# Autodesk Inventor assembly: GP6-100
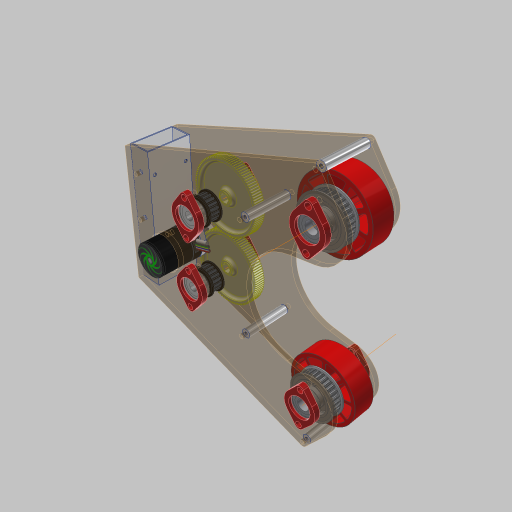
[picture p0: Inventor's stored thumbnail of the model, 512x512]
Saved by Autodesk Inventor 2023.5 (Build 275446000, 446)
## iProperties
Created: 2025-02-23
Part Number: GP6-100
Document SubType Name: Assembly
Designer: slick
Author: slick
## Documents named in this file (16)
- C:\Users\slick\OneDrive\Desktop\2025-ReefScape---CAD\Gripper\GP6\GP6-100.iam
- C:\Users\slick\OneDrive\Desktop\2025-ReefScape---CAD\Gripper\GP6\GP6-001.ipt
- C:\Users\slick\OneDrive\Desktop\2025-ReefScape---CAD\Gripper\GP6\GP6-003.ipt
- C:\Users\slick\OneDrive\Desktop\2025-ReefScape---CAD\Gripper\GP6\GP6-002.ipt
- C:\Users\slick\OneDrive\Desktop\2025-ReefScape---CAD\COMMON PARTS\BEARINGS\0_500_ID_x_1_125_OD_x_0_313_WD_Flanged_Bearing_217-2731.ipt
- C:\Users\slick\OneDrive\Desktop\2025-ReefScape---CAD\COMMON PARTS\BEARINGS\Bearing Retainer\Retainer.ipt
- C:\Users\slick\OneDrive\Desktop\2025-ReefScape---CAD\COMMON PARTS\BEARINGS\0_375_ID_x_1_125_OD_x_0_313_WD_Flanged_Bearing_217-2732.ipt
- C:\Users\slick\OneDrive\Desktop\2025-ReefScape---CAD\Gripper\GP6\GP6-005.ipt
- C:\Users\slick\OneDrive\Desktop\2025-ReefScape---CAD\COMMON PARTS\MOTORS\Minion.ipt
- C:\Users\slick\OneDrive\Desktop\2025-ReefScape---CAD\Gripper\GP6\GP6-006.ipt
- C:\Users\slick\OneDrive\Desktop\2025-ReefScape---CAD\COMMON PARTS\GEARS\15t Spur Gear\15t Spur Gear.ipt
- C:\Users\slick\OneDrive\Desktop\2025-ReefScape---CAD\COMMON PARTS\GEARS\32 dp gear\100t_Aluminum_Spur_Gear_32_DP_3_8_Hex_Bore_217-5865.ipt
- C:\Users\slick\OneDrive\Desktop\2025-ReefScape---CAD\Gripper\GP6\GP6-007.ipt
- C:\Users\slick\OneDrive\Desktop\2025-ReefScape---CAD\COMMON PARTS\PULLEYS\htd\30t_x_9mm_Wide_Double_Flange_Aluminum_Pulley_HTD_5mm_1_2_Hex_Bore_217-3229.ipt
- C:\Users\slick\OneDrive\Desktop\2025-ReefScape---CAD\COMMON PARTS\PULLEYS\htd\18t_x_9mm_Wide_Double_Flange_Aluminum_Pulley_HTD_5mm_1_2_Hex_Bore_217-3225.ipt
- C:\Users\slick\OneDrive\Desktop\2025-ReefScape---CAD\COMMON PARTS\WHEELS\am-3946 3IN 375Hex Compliant Wheel REV 3.ipt
## Components (35 placed, 15 different names)
1. GP6-001:1 — Insert:1, Insert:2, Insert:35, Insert:36, Insert:41, Insert:42, Insert:43, Insert:46, Insert:47, Insert:54, Insert:55, Insert:60, Insert:61, Insert:62, Insert:63
2. GP6-003:1 — Insert:1, Insert:2, Insert:3, Insert:4
3. GP6-002:1 — Insert:3, Insert:4, Insert:38, Insert:39, Insert:40, Insert:44, Insert:45, Insert:48, Insert:49, Insert:50, Insert:51, Insert:52, Insert:53, Insert:56, Insert:57, Insert:58, Insert:59
4. GP6-005:1 — Insert:31, Insert:32, Insert:33, Insert:34
5. Minion:1 — Insert:31, Insert:32, Insert:37
6. GP6-006:1 — Insert:33, Insert:35
7. GP6-006:2 — Insert:34, Insert:36
8. 15t Spur Gear:1 — Insert:37
9. 100t_Aluminum_Spur_Gear_32_DP_3_8_Hex_Bore_217-5865:1 — Flush:1, Mate:12, Mate:15
10. 100t_Aluminum_Spur_Gear_32_DP_3_8_Hex_Bore_217-5865:2 — Flush:1, Mate:14
11. GP6-007:1 — Insert:38
12. GP6-007:2 — Insert:40
13. GP6-007:3 — Insert:41
14. GP6-007:4 — Insert:39
15. 30t_x_9mm_Wide_Double_Flange_Aluminum_Pulley_HTD_5mm_1_2_Hex_Bore_217-3229:1 — Flush:2, Flush:4, Mate:9, Mate:10
16. 30t_x_9mm_Wide_Double_Flange_Aluminum_Pulley_HTD_5mm_1_2_Hex_Bore_217-3229:2 — Flush:3, Flush:4, Mate:17, Mate:18
17. 18t_x_9mm_Wide_Double_Flange_Aluminum_Pulley_HTD_5mm_1_2_Hex_Bore_217-3225:1 — Flush:2, Mate:11, Mate:12
18. 18t_x_9mm_Wide_Double_Flange_Aluminum_Pulley_HTD_5mm_1_2_Hex_Bore_217-3225:2 — Flush:3, Mate:13, Mate:14, Mate:16
19. am-3946 3IN 375Hex Compliant Wheel REV 3:1 — Mate:9, Flush:5
20. am-3946 3IN 375Hex Compliant Wheel REV 3:4 — Mate:18, Flush:5
21. 0_500_ID_x_1_125_OD_x_0_313_WD_Flanged_Bearing_217-2731:1 — Insert:45, Mate:10
22. 0_500_ID_x_1_125_OD_x_0_313_WD_Flanged_Bearing_217-2731:2 — Insert:42
23. 0_500_ID_x_1_125_OD_x_0_313_WD_Flanged_Bearing_217-2731:3 — Insert:43
24. 0_500_ID_x_1_125_OD_x_0_313_WD_Flanged_Bearing_217-2731:4 — Insert:44, Mate:17
25. 0_375_ID_x_1_125_OD_x_0_313_WD_Flanged_Bearing_217-2732:1 — Insert:46, Mate:15
26. 0_375_ID_x_1_125_OD_x_0_313_WD_Flanged_Bearing_217-2732:2 — Insert:49, Mate:11
27. 0_375_ID_x_1_125_OD_x_0_313_WD_Flanged_Bearing_217-2732:3 — Insert:48, Mate:13, Mate:16
28. 0_375_ID_x_1_125_OD_x_0_313_WD_Flanged_Bearing_217-2732:4 — Insert:47
29. Retainer:1 — Insert:50, Insert:51
30. Retainer:2 — Insert:52, Insert:53
31. Retainer:3 — Insert:54, Insert:55
32. Retainer:4 — Insert:56, Insert:57
33. Retainer:5 — Insert:58, Insert:59
34. Retainer:6 — Insert:62, Insert:63
35. Retainer:7 — Insert:60, Insert:61
## Relationships (52: Insert 37, Mate 10, Flush 5)
- Insert:1: GP6-001:1 ↔ GP6-003:1
- Insert:2: GP6-001:1 ↔ GP6-003:1
- Insert:3: GP6-003:1 ↔ GP6-002:1
- Insert:4: GP6-003:1 ↔ GP6-002:1
- Insert:31: GP6-005:1 ↔ Minion:1
- Insert:32: GP6-005:1 ↔ Minion:1
- Insert:33: GP6-005:1 ↔ GP6-006:1
- Insert:34: GP6-005:1 ↔ GP6-006:2
- Insert:35: GP6-001:1 ↔ GP6-006:1
- Insert:36: GP6-001:1 ↔ GP6-006:2
- Insert:37: Minion:1 ↔ 15t Spur Gear:1
- Flush:1: 100t_Aluminum_Spur_Gear_32_DP_3_8_Hex_Bore_217-5865:1 ↔ 100t_Aluminum_Spur_Gear_32_DP_3_8_Hex_Bore_217-5865:2
- Insert:38: GP6-002:1 ↔ GP6-007:1
- Insert:39: GP6-002:1 ↔ GP6-007:4
- Insert:40: GP6-002:1 ↔ GP6-007:2
- Insert:41: GP6-001:1 ↔ GP6-007:3
- Flush:2: 30t_x_9mm_Wide_Double_Flange_Aluminum_Pulley_HTD_5mm_1_2_Hex_Bore_217-3229:1 ↔ 18t_x_9mm_Wide_Double_Flange_Aluminum_Pulley_HTD_5mm_1_2_Hex_Bore_217-3225:1
- Flush:3: 30t_x_9mm_Wide_Double_Flange_Aluminum_Pulley_HTD_5mm_1_2_Hex_Bore_217-3229:2 ↔ 18t_x_9mm_Wide_Double_Flange_Aluminum_Pulley_HTD_5mm_1_2_Hex_Bore_217-3225:2
- Flush:4: 30t_x_9mm_Wide_Double_Flange_Aluminum_Pulley_HTD_5mm_1_2_Hex_Bore_217-3229:1 ↔ 30t_x_9mm_Wide_Double_Flange_Aluminum_Pulley_HTD_5mm_1_2_Hex_Bore_217-3229:2
- Mate:9: 30t_x_9mm_Wide_Double_Flange_Aluminum_Pulley_HTD_5mm_1_2_Hex_Bore_217-3229:1 ↔ am-3946 3IN 375Hex Compliant Wheel REV 3:1
- Insert:42: GP6-001:1 ↔ 0_500_ID_x_1_125_OD_x_0_313_WD_Flanged_Bearing_217-2731:2
- Insert:43: GP6-001:1 ↔ 0_500_ID_x_1_125_OD_x_0_313_WD_Flanged_Bearing_217-2731:3
- Insert:44: GP6-002:1 ↔ 0_500_ID_x_1_125_OD_x_0_313_WD_Flanged_Bearing_217-2731:4
- Insert:45: GP6-002:1 ↔ 0_500_ID_x_1_125_OD_x_0_313_WD_Flanged_Bearing_217-2731:1
- Insert:46: GP6-001:1 ↔ 0_375_ID_x_1_125_OD_x_0_313_WD_Flanged_Bearing_217-2732:1
- Insert:47: GP6-001:1 ↔ 0_375_ID_x_1_125_OD_x_0_313_WD_Flanged_Bearing_217-2732:4
- Insert:48: GP6-002:1 ↔ 0_375_ID_x_1_125_OD_x_0_313_WD_Flanged_Bearing_217-2732:3
- Insert:49: GP6-002:1 ↔ 0_375_ID_x_1_125_OD_x_0_313_WD_Flanged_Bearing_217-2732:2
- Insert:50: GP6-002:1 ↔ Retainer:1
- Insert:51: GP6-002:1 ↔ Retainer:1
- Insert:52: GP6-002:1 ↔ Retainer:2
- Insert:53: GP6-002:1 ↔ Retainer:2
- Insert:54: GP6-001:1 ↔ Retainer:3
- Insert:55: GP6-001:1 ↔ Retainer:3
- Insert:56: GP6-002:1 ↔ Retainer:4
- Insert:57: GP6-002:1 ↔ Retainer:4
- Insert:58: GP6-002:1 ↔ Retainer:5
- Insert:59: GP6-002:1 ↔ Retainer:5
- Insert:60: GP6-001:1 ↔ Retainer:7
- Insert:61: GP6-001:1 ↔ Retainer:7
- Insert:62: GP6-001:1 ↔ Retainer:6
- Insert:63: GP6-001:1 ↔ Retainer:6
- Mate:10: 30t_x_9mm_Wide_Double_Flange_Aluminum_Pulley_HTD_5mm_1_2_Hex_Bore_217-3229:1 ↔ 0_500_ID_x_1_125_OD_x_0_313_WD_Flanged_Bearing_217-2731:1
- Mate:11: 18t_x_9mm_Wide_Double_Flange_Aluminum_Pulley_HTD_5mm_1_2_Hex_Bore_217-3225:1 ↔ 0_375_ID_x_1_125_OD_x_0_313_WD_Flanged_Bearing_217-2732:2
- Mate:12: 100t_Aluminum_Spur_Gear_32_DP_3_8_Hex_Bore_217-5865:1 ↔ 18t_x_9mm_Wide_Double_Flange_Aluminum_Pulley_HTD_5mm_1_2_Hex_Bore_217-3225:1
- Mate:13: 18t_x_9mm_Wide_Double_Flange_Aluminum_Pulley_HTD_5mm_1_2_Hex_Bore_217-3225:2 ↔ 0_375_ID_x_1_125_OD_x_0_313_WD_Flanged_Bearing_217-2732:3
- Mate:14: 100t_Aluminum_Spur_Gear_32_DP_3_8_Hex_Bore_217-5865:2 ↔ 18t_x_9mm_Wide_Double_Flange_Aluminum_Pulley_HTD_5mm_1_2_Hex_Bore_217-3225:2
- Mate:15 (3.175 mm): 100t_Aluminum_Spur_Gear_32_DP_3_8_Hex_Bore_217-5865:1 ↔ 0_375_ID_x_1_125_OD_x_0_313_WD_Flanged_Bearing_217-2732:1
- Mate:16 (3.175 mm): 18t_x_9mm_Wide_Double_Flange_Aluminum_Pulley_HTD_5mm_1_2_Hex_Bore_217-3225:2 ↔ 0_375_ID_x_1_125_OD_x_0_313_WD_Flanged_Bearing_217-2732:3
- Mate:17: 30t_x_9mm_Wide_Double_Flange_Aluminum_Pulley_HTD_5mm_1_2_Hex_Bore_217-3229:2 ↔ 0_500_ID_x_1_125_OD_x_0_313_WD_Flanged_Bearing_217-2731:4
- Mate:18: 30t_x_9mm_Wide_Double_Flange_Aluminum_Pulley_HTD_5mm_1_2_Hex_Bore_217-3229:2 ↔ am-3946 3IN 375Hex Compliant Wheel REV 3:4
- Flush:5: am-3946 3IN 375Hex Compliant Wheel REV 3:1 ↔ am-3946 3IN 375Hex Compliant Wheel REV 3:4
